# Autodesk Inventor assembly: Assembly_Cube_Z-Stage_manual
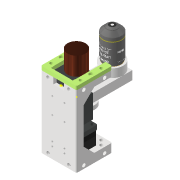
[picture p0: Inventor's stored thumbnail of the model, 180x180]
Saved by Autodesk Inventor 2022 (Build 260153000, 153)
## iProperties
Created: 2023-02-17
Part Number: Assembly_Cube_Z-Stage_manual
Document SubType Name: Assembly
Designer: diederichbenedict
Author: diederichbenedict
## Documents named in this file (9)
- C:\Users\diederichbenedict\Dropbox\Dokumente\Promotion\PROJECTS\openUC2-CAD\INVENTOR\Assembly_Cube_Z-Stage_manual.iam
- C:\Users\diederichbenedict\Dropbox\Dokumente\Promotion\PROJECTS\openUC2-CAD\INVENTOR\00_Microscope_objective_10x.ipt
- C:\Users\diederichbenedict\Dropbox\Dokumente\Promotion\PROJECTS\openUC2-CAD\INVENTOR\30_Linear_Stage_NEMA11_China_base_universal_v3.ipt
- C:\Users\diederichbenedict\Dropbox\Dokumente\Promotion\PROJECTS\openUC2-CAD\INVENTOR\00_JST_4x_200mm.ipt
- C:\Users\diederichbenedict\Dropbox\Dokumente\Promotion\PROJECTS\openUC2-CAD\INVENTOR\30_Linear_Stage_NEMA11_arm_bayonetmount_femalemale.ipt
- C:\Users\diederichbenedict\Dropbox\Dokumente\Promotion\PROJECTS\openUC2-CAD\INVENTOR\30_Linear_Stage_NEMA11_baseholder_bayonetmount_25mmFiltermount.ipt
- C:\Users\diederichbenedict\Dropbox\Dokumente\Promotion\PROJECTS\openUC2-CAD\INVENTOR\30_Linear_Stage_NEMA11_baseholder_bayonetmount_objective_v0.ipt
- C:\Users\diederichbenedict\Dropbox\Dokumente\Promotion\PROJECTS\openUC2-CAD\INVENTOR\30_Linear_Stage_NEMA11_China_lid_universal_extender_v2.ipt
- C:\Users\diederichbenedict\Dropbox\Dokumente\Promotion\PROJECTS\openUC2-CAD\INVENTOR\00_Linear_Stage_Manual_50mm_china.iam
## Components (8 placed, 8 different names)
1. 00_Linear_Stage_Manual_50mm_china:1 [sub-assembly] — Passend:1, Winkel:1, Fluchtend:1, Passend:2, Fluchtend:6, Insert:11, Insert:12
2. 30_Linear_Stage_NEMA11_China_base_universal_v3:1 — Passend:2, Fluchtend:6, Insert:10, Angle:2
3. 00_Microscope_objective_10x:1 — Einfügen:9
4. 00_JST_4x_200mm:1
5. 30_Linear_Stage_NEMA11_baseholder_bayonetmount_25mmFiltermount:1 — Einfügen:9, Insert:13
6. 30_Linear_Stage_NEMA11_baseholder_bayonetmount_objective_v0:1
7. 30_Linear_Stage_NEMA11_China_lid_universal_extender_v2:1 — Insert:10, Angle:2
8. 30_Linear_Stage_NEMA11_arm_bayonetmount_femalemale:1 — Insert:11, Insert:12, Insert:13
## Relationships (11: Insert 5, Mate 2, Angle 2, Flush 2)
- Passend:1 [Mate]: 00_Linear_Stage_Manual_50mm_china:1
- Winkel:1 [Angle] (0 deg): 00_Linear_Stage_Manual_50mm_china:1
- Fluchtend:1 [Flush]: 00_Linear_Stage_Manual_50mm_china:1
- Passend:2 [Mate]: 00_Linear_Stage_Manual_50mm_china:1 ↔ 30_Linear_Stage_NEMA11_China_base_universal_v3:1
- Fluchtend:6 [Flush]: 00_Linear_Stage_Manual_50mm_china:1 ↔ 30_Linear_Stage_NEMA11_China_base_universal_v3:1
- Einfügen:9 [Insert]: 00_Microscope_objective_10x:1 ↔ 30_Linear_Stage_NEMA11_baseholder_bayonetmount_25mmFiltermount:1
- Insert:10: 30_Linear_Stage_NEMA11_China_base_universal_v3:1 ↔ 30_Linear_Stage_NEMA11_China_lid_universal_extender_v2:1
- Angle:2 (0 deg): 30_Linear_Stage_NEMA11_China_base_universal_v3:1 ↔ 30_Linear_Stage_NEMA11_China_lid_universal_extender_v2:1
- Insert:11: 00_Linear_Stage_Manual_50mm_china:1 ↔ 30_Linear_Stage_NEMA11_arm_bayonetmount_femalemale:1
- Insert:12: 00_Linear_Stage_Manual_50mm_china:1 ↔ 30_Linear_Stage_NEMA11_arm_bayonetmount_femalemale:1
- Insert:13: 30_Linear_Stage_NEMA11_baseholder_bayonetmount_25mmFiltermount:1 ↔ 30_Linear_Stage_NEMA11_arm_bayonetmount_femalemale:1
